# Autodesk Inventor assembly: Intake
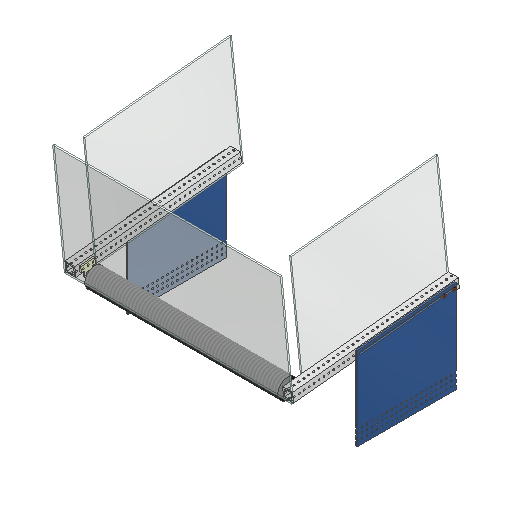
[picture p0: Inventor's stored thumbnail of the model, 512x512]
Saved by Autodesk Inventor 2025.3 (Build 293356000, 356)
## iProperties
Created: 2026-05-13
Part Number: Intake
Document SubType Name: Assembly
Designer: djair.oliveira
Author: djair.oliveira
## Documents named in this file (8)
- C:\Users\djair.oliveira\Documents\GitHub\MT_2026\CAD\Model B\Intake\Intake.iam
- C:\Users\djair.oliveira\Documents\GitHub\MT_2026\CAD\Model B\Intake\Guia - Intake.ipt
- C:\Users\djair.oliveira\Documents\GitHub\MT_2026\CAD\Model B\Intake\Move - Intake.ipt
- C:\Users\djair.oliveira\Documents\GitHub\MT_2026\CAD\Model B\Intake\Suporte Guia - Intake.ipt
- C:\Users\djair.oliveira\Documents\GitHub\MT_2026\CAD\Model B\Intake\Suporte Coletor - Intake.ipt
- C:\Users\djair.oliveira\Documents\GitHub\MT_2026\CAD\Model B\Intake\Coletor - Intake.ipt
- C:\Users\djair.oliveira\Documents\GitHub\MT_2026\CAD\Model B\Intake\Chapa Frontal - Intake.ipt
- C:\Users\djair.oliveira\Documents\GitHub\MT_2026\CAD\Model B\Intake\Chapa Lateral - Intake.ipt
## Components (14 placed, 7 different names)
1. Guia - Intake:1 — Coincidente:1, Coincidente:2, Coincidente:3, Coincidente:5
2. Guia - Intake:2 — Coincidente:1, Coincidente:2, Coincidente:3, Coincidente:4, Tangente:1, Tangente:2, Tangente:3
3. Move - Intake:1 — Coincidente:5, Coincidente:6, Coincidente:7, Coincidente:8, Coincidente:9, Coincidente:10, Coincidente:11, Coincidente:16, Coincidente:17, Coincidente:18, Coincidente:26, Alinhado:3, Alinhado:4
4. Move - Intake:2 — Coincidente:4, Tangente:1, Tangente:2, Tangente:3, Coincidente:6, Coincidente:7, Coincidente:12, Coincidente:13, Coincidente:14, Coincidente:15, Coincidente:19, Coincidente:20, Coincidente:21, Coincidente:24, Alinhado:1, Alinhado:2, Coincidente:25, Alinhado:5, Alinhado:6
5. Suporte Guia - Intake:1 — Coincidente:8, Coincidente:9
6. Suporte Guia - Intake:2 — Coincidente:14, Coincidente:15
7. Suporte Guia - Intake:3 — Coincidente:12, Coincidente:13
8. Suporte Guia - Intake:4 — Coincidente:10, Coincidente:11
9. Suporte Coletor - Intake:1 — Coincidente:19, Coincidente:20, Coincidente:21, Coincidente:22, Coincidente:23
10. Suporte Coletor - Intake:2 — Coincidente:16, Coincidente:17, Coincidente:18
11. Coletor - Intake:1 — Coincidente:22, Coincidente:23
12. Chapa Frontal - Intake:1 — Coincidente:24, Alinhado:1, Alinhado:2
13. Chapa Lateral - Intake:1 — Coincidente:26, Alinhado:3, Alinhado:4
14. Chapa Lateral - Intake:2 — Coincidente:25, Alinhado:5, Alinhado:6
## Relationships (35: Mate 26, Flush 6, Tangent 3)
- Coincidente:1 [Mate] (584.2 mm): Guia - Intake:1 ↔ Guia - Intake:2
- Coincidente:2 [Mate]: Guia - Intake:1 ↔ Guia - Intake:2
- Coincidente:3 [Mate]: Guia - Intake:1 ↔ Guia - Intake:2
- Coincidente:4 [Mate]: Guia - Intake:2 ↔ Move - Intake:2
- Tangente:1 (-5.5 mm): Guia - Intake:2 ↔ Move - Intake:2
- Tangente:2 (-5.5 mm): Guia - Intake:2 ↔ Move - Intake:2
- Tangente:3 (4 mm): Guia - Intake:2 ↔ Move - Intake:2
- Coincidente:5 [Mate]: Guia - Intake:1 ↔ Move - Intake:1
- Coincidente:6 [Mate]: Move - Intake:1 ↔ Move - Intake:2
- Coincidente:7 [Mate]: Move - Intake:1 ↔ Move - Intake:2
- Coincidente:8 [Mate]: Move - Intake:1 ↔ Suporte Guia - Intake:1
- Coincidente:9 [Mate]: Move - Intake:1 ↔ Suporte Guia - Intake:1
- Coincidente:10 [Mate]: Move - Intake:1 ↔ Suporte Guia - Intake:4
- Coincidente:11 [Mate]: Move - Intake:1 ↔ Suporte Guia - Intake:4
- Coincidente:12 [Mate]: Move - Intake:2 ↔ Suporte Guia - Intake:3
- Coincidente:13 [Mate]: Move - Intake:2 ↔ Suporte Guia - Intake:3
- Coincidente:14 [Mate]: Move - Intake:2 ↔ Suporte Guia - Intake:2
- Coincidente:15 [Mate]: Move - Intake:2 ↔ Suporte Guia - Intake:2
- Coincidente:16 [Mate]: Move - Intake:1 ↔ Suporte Coletor - Intake:2
- Coincidente:17 [Mate]: Move - Intake:1 ↔ Suporte Coletor - Intake:2
- Coincidente:18 [Mate]: Move - Intake:1 ↔ Suporte Coletor - Intake:2
- Coincidente:19 [Mate]: Move - Intake:2 ↔ Suporte Coletor - Intake:1
- Coincidente:20 [Mate]: Move - Intake:2 ↔ Suporte Coletor - Intake:1
- Coincidente:21 [Mate]: Move - Intake:2 ↔ Suporte Coletor - Intake:1
- Coincidente:22 [Mate]: Suporte Coletor - Intake:1 ↔ Coletor - Intake:1
- Coincidente:23 [Mate]: Suporte Coletor - Intake:1 ↔ Coletor - Intake:1
- Coincidente:24 [Mate]: Move - Intake:2 ↔ Chapa Frontal - Intake:1
- Alinhado:1 [Flush]: Move - Intake:2 ↔ Chapa Frontal - Intake:1
- Alinhado:2 [Flush]: Move - Intake:2 ↔ Chapa Frontal - Intake:1
- Coincidente:25 [Mate]: Move - Intake:2 ↔ Chapa Lateral - Intake:2
- Coincidente:26 [Mate]: Move - Intake:1 ↔ Chapa Lateral - Intake:1
- Alinhado:3 [Flush]: Move - Intake:1 ↔ Chapa Lateral - Intake:1
- Alinhado:4 [Flush]: Move - Intake:1 ↔ Chapa Lateral - Intake:1
- Alinhado:5 [Flush]: Move - Intake:2 ↔ Chapa Lateral - Intake:2
- Alinhado:6 [Flush]: Move - Intake:2 ↔ Chapa Lateral - Intake:2
